# Autodesk Inventor assembly: Stift_symmetrieebene
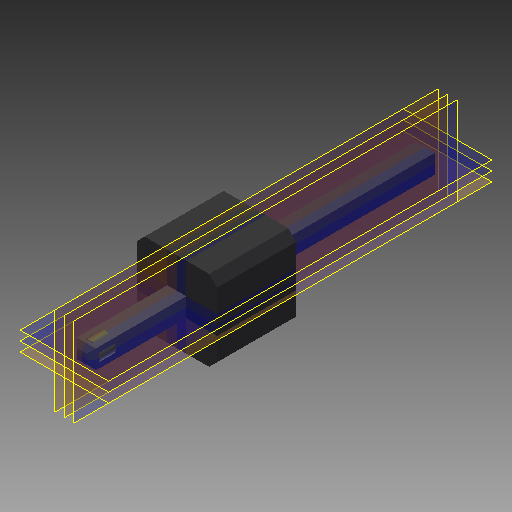
[picture p0: Inventor's stored thumbnail of the model, 512x512]
Saved by Autodesk Inventor 2017.3 (Build 213257000, 257)
## iProperties
Part Number: Stift_symmetrieebene
Material: Generisch
Document SubType Name: Assembly
Designer: Enno
Author: Enno
## Documents named in this file (2)
- C:\Users\Enno-LT\Desktop\IMU_Motion_Classification\Casing\Stiftleiste\Män\Gerade\Stift_symmetrieebene.iam
- C:\Users\Enno-LT\Desktop\IMU_Motion_Classification\Casing\Stiftleiste\Män\Gerade\Stiftleiste_Male.ipt
## Components (1 placed, 1 different names)
1. Stiftleiste_Male:1 — Passend:1, Winkel:1, Passend:2, Winkel:2, Passend:3, Winkel:3, Passend:4, Winkel:4
## Relationships (10: Mate 4, Angle 4, Symmetry 2)
- Passend:1 [Mate]: Stiftleiste_Male:1
- Winkel:1 [Angle] (0 deg): Stiftleiste_Male:1
- Passend:2 [Mate]: Stiftleiste_Male:1
- Winkel:2 [Angle] (90 deg): Stiftleiste_Male:1
- Symmetrie:1
- Passend:3 [Mate]: Stiftleiste_Male:1
- Winkel:3 [Angle] (90 deg): Stiftleiste_Male:1
- Passend:4 [Mate]: Stiftleiste_Male:1
- Winkel:4 [Angle] (90 deg): Stiftleiste_Male:1
- Symmetrie:2
